# Autodesk Inventor assembly: Wheel
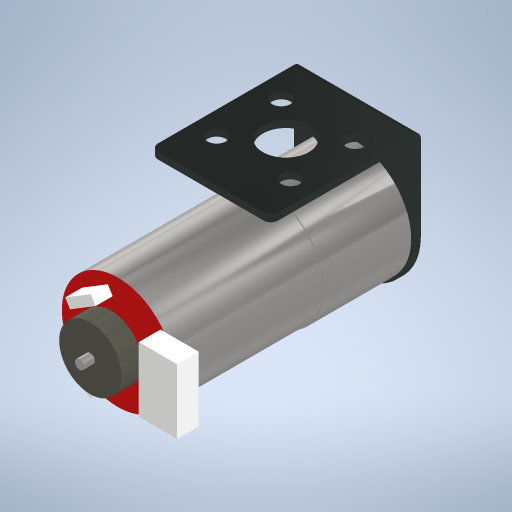
[picture p0: Inventor's stored thumbnail of the model, 512x512]
Saved by Autodesk Inventor 2024.2 (Build 282272000, 272)
## iProperties
Created: 2025-06-30
Part Number: Wheel
Document SubType Name: Assembly
Designer: Admin
Author: Admin
## Documents named in this file (3)
- C:\Users\Admin\Documents\GitHub\ExplorateurErrant\Assemblies\Wheel.iam
- C:\Users\Admin\Documents\GitHub\ExplorateurErrant\Motors\DC-JGA25\WH-Bracket-JGA25.ipt
- C:\Users\Admin\Documents\GitHub\ExplorateurErrant\Motors\DC-JGA25\WH-Motor-JGA25.ipt
## Components (2 placed, 2 different names)
1. WH-Bracket-JGA25:1 — Mate:1, Mate:2, Mate:3
2. WH-Motor-JGA25:1 — Mate:1, Mate:2, Mate:3
## Relationships (3: Mate 3)
- Mate:1: WH-Bracket-JGA25:1 ↔ WH-Motor-JGA25:1
- Mate:2: WH-Bracket-JGA25:1 ↔ WH-Motor-JGA25:1
- Mate:3: WH-Bracket-JGA25:1 ↔ WH-Motor-JGA25:1
